# Autodesk Inventor assembly: base wheel
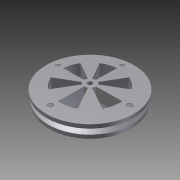
[picture p0: Inventor's stored thumbnail of the model, 180x180]
Saved by Autodesk Inventor 2011 (Build 150239000, 239)
## iProperties
Created: 2010-04-18
Part Number: base wheel
Document SubType Name: Assembly
Designer: lucio
Author: lucio
## Documents named in this file (4)
- C:\Users\lucio\Documents\Inventor\caterpillar\base wheel.iam
- C:\Users\lucio\Documents\Inventor\caterpillar\wheel.ipt
- C:\Users\lucio\Documents\Inventor\Content Center Files\R2011\en-US\ANSI B18.3.1M(5)\ANSI B18.3.1M - M4x0.7 x 16(3).ipt
- C:\Users\lucio\Documents\Inventor\Content Center Files\R2011\en-US\ANSI B 18.2.4.1 M(1)\ANSI B 18.2.4.1 M - M4 x 0.7Style 2.ipt
## Components (10 placed, 3 different names)
1. wheel:1 — Mate:1, Mate:2, Mate:3, Insert:1, Insert:2, Insert:3, Insert:4
2. wheel:2 — Mate:1, Mate:2, Mate:3, Insert:5, Insert:6, Insert:7, Insert:8
3. Drilled Forged Hexagon Socket Head Cap Screw - 6 Holes - Metric M4x0.7 x 16:1 — Insert:4
4. Drilled Forged Hexagon Socket Head Cap Screw - 6 Holes - Metric M4x0.7 x 16:2 — Insert:3
5. Drilled Forged Hexagon Socket Head Cap Screw - 6 Holes - Metric M4x0.7 x 16:3 — Insert:2
6. Drilled Forged Hexagon Socket Head Cap Screw - 6 Holes - Metric M4x0.7 x 16:4 — Insert:1
7. Hex Nut Metric M4 x 0.7:1 — Insert:8
8. Hex Nut Metric M4 x 0.7:2 — Insert:7
9. Hex Nut Metric M4 x 0.7:3 — Insert:5
10. Hex Nut Metric M4 x 0.7:4 — Insert:6
## Relationships (11: Insert 8, Mate 3)
- Mate:1: wheel:1 ↔ wheel:2
- Mate:2: wheel:1 ↔ wheel:2
- Mate:3: wheel:1 ↔ wheel:2
- Insert:1: wheel:1 ↔ Drilled Forged Hexagon Socket Head Cap Screw - 6 Holes - Metric M4x0.7 x 16:4
- Insert:2: wheel:1 ↔ Drilled Forged Hexagon Socket Head Cap Screw - 6 Holes - Metric M4x0.7 x 16:3
- Insert:3: wheel:1 ↔ Drilled Forged Hexagon Socket Head Cap Screw - 6 Holes - Metric M4x0.7 x 16:2
- Insert:4: wheel:1 ↔ Drilled Forged Hexagon Socket Head Cap Screw - 6 Holes - Metric M4x0.7 x 16:1
- Insert:5: wheel:2 ↔ Hex Nut Metric M4 x 0.7:3
- Insert:6: wheel:2 ↔ Hex Nut Metric M4 x 0.7:4
- Insert:7: wheel:2 ↔ Hex Nut Metric M4 x 0.7:2
- Insert:8: wheel:2 ↔ Hex Nut Metric M4 x 0.7:1
